# Autodesk Inventor assembly: Ball Intake
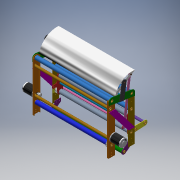
[picture p0: Inventor's stored thumbnail of the model, 180x180]
Saved by Autodesk Inventor 2017 (Build 210142000, 142)
## iProperties
Created: 2017-01-13
Part Number: Ball Intake
Document SubType Name: Assembly
Designer: Ben
Author: Ben
## Documents named in this file (27)
- C:\Users\Ben\Desktop\Projects\2017 Robot\Ball Intake\Ball Intake.iam
- C:\Users\Ben\Desktop\Projects\2017 Robot\Ball Intake\Front Plate.ipt
- C:\Users\Ben\Desktop\Projects\2017 Robot\Ball Intake\Churro Cross Brace.ipt
- C:\Users\Ben\Desktop\Projects\2017 Robot\Ball Intake\Back Plate.ipt
- C:\Users\Ben\Desktop\Projects\2017 Robot\Ball Intake\Cross Plate.ipt
- C:\Users\Ben\Desktop\Projects\2017 Robot\Ball Intake\Roller Assembly.iam
- C:\Users\Ben\Desktop\Projects\2017 Robot\Ball Intake\Swing Arm.ipt
- C:\Users\Ben\Desktop\Projects\2017 Robot\Ball Intake\Rear roller plate.ipt
- C:\Users\Ben\Desktop\Projects\2017 Robot\Ball Intake\Hopper pully plate.ipt
- C:\Users\Ben\Desktop\Projects\2017 Robot\Ball Intake\Flipper Plate.ipt
- C:\Users\Ben\Desktop\Projects\2017 Robot\Ball Intake\Kick Plate.ipt
- C:\Users\Ben\Desktop\Projects\2017 Robot\Ball Intake\Shorter Churro Cross Brace.ipt
- C:\Users\Ben\Desktop\Projects\2017 Robot\Ball Intake\Hopper roller assembly.iam
- C:\Users\Ben\Desktop\Projects\2017 Robot\Ball Intake\Hopper roller rear assembly.iam
- C:\Users\Ben\Desktop\Projects\2017 Robot\Ball Intake\Front Idler roller assembly.iam
- C:\Users\Ben\Desktop\Projects\2017 Robot\Ball Intake\Mini CIM.ipt
- C:\Users\Ben\Desktop\Projects\2017 Robot\Ball Intake\.375 bearing.ipt
- C:\Users\Ben\Desktop\Projects\2017 Robot\Ball Intake\Front C Left.ipt
- C:\Users\Ben\Desktop\Projects\2017 Robot\Ball Intake\.25 bushing.ipt
- C:\Users\Ben\Desktop\Projects\2017 Robot\Ball Intake\XL 24T Pulley.ipt
- C:\Users\Ben\Desktop\Projects\2017 Robot\Ball Intake\XL 12T Timing Pulley.ipt
- C:\Users\Ben\Desktop\Projects\2017 Robot\Ball Intake\1in Short PVC Roller.ipt
- C:\Users\Ben\Desktop\Projects\2017 Robot\Ball Intake\Bottom Roller.ipt
- C:\Users\Ben\Desktop\Projects\2017 Robot\Ball Intake\Roller End Plug.ipt
- C:\Users\Ben\Desktop\Projects\2017 Robot\Ball Intake\Intake Roller.ipt
- C:\Users\Ben\Desktop\Projects\2017 Robot\Ball Intake\Tie Rod 2.ipt
- C:\Users\Ben\Desktop\Projects\2017 Robot\Ball Intake\Cross Brace.ipt
## Components (73 placed, 26 different names)
1. Front Plate:2 — Flush:2, Insert:10, Flush:6, Flush:17, Flush:18, Mate:10, Insert:46, Insert:55, Insert:56, Insert:82, Mate:14, Flush:22, Flush:23, Insert:113, Mate:17, Angle:1
2. Back Plate:1 — Insert:5, Insert:13, Mate:3, Flush:8, Mate:6, Insert:28, Flush:9, Flush:19, Insert:130, Insert:131, Insert:142, Insert:143
3. Back Plate:2 — Flush:2, Insert:7, Flush:6, Insert:25, Mate:4, Flush:7, Mate:5, Insert:27, Flush:10, Flush:17, Flush:19, Insert:115, Insert:117, Insert:140, Insert:141
4. Churro Cross Brace:3 — Insert:5, Insert:7
5. Cross Plate:1 — Insert:10, Insert:25, Mate:7, Mate:12, Flush:20
6. Cross Plate:2 — Insert:13, Mate:8, Flush:21
7. Roller Assembly:4 [sub-assembly] — Insert:118
8. Swing Arm:1 — Insert:39, Insert:60, Insert:66, Insert:135, Insert:137, Angle:1, Insert:139
9. Swing Arm:2 — Insert:71, Insert:75
10. Rear roller plate:3 — Mate:3, Flush:8, Mate:6, Insert:67
11. Rear roller plate:4 — Mate:4, Flush:7, Mate:5, Insert:63
12. Hopper pully plate:1 — Insert:27, Flush:10, Insert:61, Insert:62, Insert:64
13. Hopper pully plate:2 — Insert:28, Flush:9, Insert:74, Insert:76, Insert:77
14. Flipper Plate:1 — Mate:7, Flush:14, Insert:31, Mate:12, Flush:20, Insert:89
15. Flipper Plate:2 — Mate:8, Flush:14, Flush:21, Insert:90
16. Kick Plate:1 — Insert:31, Mate:21, Insert:138
17. Shorter Churro Cross Brace:1 — Insert:39
18. Hopper roller assembly:1 [sub-assembly] — Insert:124
19. Hopper roller rear assembly:1 [sub-assembly] — Insert:123
20. Front Idler roller assembly:1 [sub-assembly] — Insert:133
21. Front Idler roller assembly:2 [sub-assembly] — Insert:122
22. Mini CIM:1 — Insert:46, Insert:94, Mate:17
23. Mini CIM:2 — Insert:87, Mate:15, Insert:95
24. Roller Assembly:5 [sub-assembly] — Insert:114
25. Roller Assembly:6 [sub-assembly] — Insert:116
26. .375 bearing:1 — Insert:63, Insert:128
27. .375 bearing:2 — Insert:55, Insert:93, Insert:121
28. .375 bearing:3 — Insert:56, Insert:122
29. .375 bearing:7 — Insert:64, Insert:123
30. .375 bearing:8 — Insert:60, Insert:132
31. .375 bearing:9 — Insert:61, Insert:135
32. .375 bearing:10 — Insert:62, Insert:124
33. .375 bearing:11 — Insert:66, Insert:127
34. .375 bearing:12 — Insert:67
35. .375 bearing:13 — Insert:84
36. .375 bearing:14 — Insert:83
37. .375 bearing:18 — Insert:77
38. .375 bearing:19 — Insert:76
39. .375 bearing:20 — Insert:74, Insert:109
40. .375 bearing:21 — Insert:75, Mate:20
41. .375 bearing:22 — Insert:71, Mate:18, Insert:136
42. .375 bearing:23 — Insert:85
43. .375 bearing:24 — Insert:82, Insert:133
44. Front C Left:1 — Mate:14, Flush:22, Flush:23, Insert:83, Insert:84, Insert:85, Insert:87, Mate:15, Insert:129
45. .25 bushing:1 — Insert:89
46. .25 bushing:2 — Insert:90
47. XL 24T Pulley:1 — Insert:93
48. XL 12T Timing Pulley:1 — Insert:94
49. XL 12T Timing Pulley:2 — Insert:95
50. 1in Short PVC Roller:1 — Insert:125, Insert:126
51. Bottom Roller:1 — Insert:99, Insert:100
52. Roller End Plug:1 — Insert:99
53. Roller End Plug:2 — Insert:100, Insert:128
54. 1in Short PVC Roller:2 — Insert:102, Insert:103
55. Roller End Plug:3 — Insert:102, Insert:132
56. Roller End Plug:4 — Insert:103, Mate:18, Insert:136
57. XL 24T Pulley:2 — Insert:109
58. .375 bearing:25 — Insert:113, Insert:114
59. .375 bearing:26 — Insert:115, Insert:116
60. .375 bearing:27 — Insert:117, Insert:118
61. Intake Roller:1 — Insert:119, Insert:120
62. Roller End Plug:5 — Insert:119, Insert:121
63. Roller End Plug:6 — Insert:120
64. Roller End Plug:7 — Insert:125, Mate:20
65. Roller End Plug:8 — Insert:126, Insert:127
66. .375 bearing:28 — Insert:129
67. .375 bearing:29 — Insert:130
68. .375 bearing:30 — Insert:131
69. Tie Rod 2:1 — Insert:137, Mate:21
70. .25 bushing:3 — Insert:138
71. .25 bushing:4 — Insert:139
72. Cross Brace:1 — Insert:140, Insert:141
73. Cross Brace:2 — Insert:142, Insert:143
## Relationships (98: Insert 69, Flush 14, Mate 14, Angle 1)
- Flush:2: Front Plate:2 ↔ Back Plate:2
- Insert:5: Back Plate:1 ↔ Churro Cross Brace:3
- Insert:7: Back Plate:2 ↔ Churro Cross Brace:3
- Insert:10: Front Plate:2 ↔ Cross Plate:1
- Insert:13: Back Plate:1 ↔ Cross Plate:2
- Flush:6: Front Plate:2 ↔ Back Plate:2
- Insert:25: Back Plate:2 ↔ Cross Plate:1
- Mate:3 (12.7 mm): Back Plate:1 ↔ Rear roller plate:3
- Mate:4 (12.7 mm): Back Plate:2 ↔ Rear roller plate:4
- Flush:7: Back Plate:2 ↔ Rear roller plate:4
- Mate:5: Back Plate:2 ↔ Rear roller plate:4
- Flush:8: Back Plate:1 ↔ Rear roller plate:3
- Mate:6: Back Plate:1 ↔ Rear roller plate:3
- Insert:27: Back Plate:2 ↔ Hopper pully plate:1
- Insert:28: Back Plate:1 ↔ Hopper pully plate:2
- Flush:9: Back Plate:1 ↔ Hopper pully plate:2
- Flush:10: Back Plate:2 ↔ Hopper pully plate:1
- Mate:7: Cross Plate:1 ↔ Flipper Plate:1
- Mate:8: Cross Plate:2 ↔ Flipper Plate:2
- Flush:14: Flipper Plate:1 ↔ Flipper Plate:2
- Insert:31 (3.175 mm): Flipper Plate:1 ↔ Kick Plate:1
- Flush:17: Front Plate:2 ↔ Back Plate:2
- Flush:18 (53.975 mm): Front Plate:2
- Mate:10 (57.658 mm): Front Plate:2
- Flush:19: Back Plate:1 ↔ Back Plate:2
- Insert:39: Swing Arm:1 ↔ Shorter Churro Cross Brace:1
- Mate:12 (61.9252 mm): Cross Plate:1 ↔ Flipper Plate:1
- Insert:46 (2.3622 mm): Front Plate:2 ↔ Mini CIM:1
- Insert:55: Front Plate:2 ↔ .375 bearing:2
- Insert:56: Front Plate:2 ↔ .375 bearing:3
- Insert:60: Swing Arm:1 ↔ .375 bearing:8
- Insert:61: Hopper pully plate:1 ↔ .375 bearing:9
- Insert:62: Hopper pully plate:1 ↔ .375 bearing:10
- Insert:63: Rear roller plate:4 ↔ .375 bearing:1
- Insert:64: Hopper pully plate:1 ↔ .375 bearing:7
- Insert:66: Swing Arm:1 ↔ .375 bearing:11
- Insert:67: Rear roller plate:3 ↔ .375 bearing:12
- Insert:71: Swing Arm:2 ↔ .375 bearing:22
- Insert:74: Hopper pully plate:2 ↔ .375 bearing:20
- Insert:75: Swing Arm:2 ↔ .375 bearing:21
- Insert:76: Hopper pully plate:2 ↔ .375 bearing:19
- Insert:77: Hopper pully plate:2 ↔ .375 bearing:18
- Insert:82: Front Plate:2 ↔ .375 bearing:24
- Flush:20: Cross Plate:1 ↔ Flipper Plate:1
- Flush:21: Cross Plate:2 ↔ Flipper Plate:2
- Mate:14 (-615.95 mm): Front Plate:2 ↔ Front C Left:1
- Flush:22: Front Plate:2 ↔ Front C Left:1
- Flush:23: Front Plate:2 ↔ Front C Left:1
- Insert:83: .375 bearing:14 ↔ Front C Left:1
- Insert:84: .375 bearing:13 ↔ Front C Left:1
- Insert:85: .375 bearing:23 ↔ Front C Left:1
- Insert:87 (2.3622 mm): Mini CIM:2 ↔ Front C Left:1
- Mate:15: Mini CIM:2 ↔ Front C Left:1
- Insert:89: Flipper Plate:1 ↔ .25 bushing:1
- Insert:90: Flipper Plate:2 ↔ .25 bushing:2
- Insert:93 (1.5875 mm): .375 bearing:2 ↔ XL 24T Pulley:1
- Insert:94 (1.5875 mm): Mini CIM:1 ↔ XL 12T Timing Pulley:1
- Insert:95 (6.35 mm): Mini CIM:2 ↔ XL 12T Timing Pulley:2
- Insert:99: Bottom Roller:1 ↔ Roller End Plug:1
- Insert:100: Bottom Roller:1 ↔ Roller End Plug:2
- Insert:102: 1in Short PVC Roller:2 ↔ Roller End Plug:3
- Insert:103: 1in Short PVC Roller:2 ↔ Roller End Plug:4
- Insert:109 (1.5875 mm): .375 bearing:20 ↔ XL 24T Pulley:2
- Insert:113: Front Plate:2 ↔ .375 bearing:25
- Insert:114 (1.5875 mm): Roller Assembly:5 ↔ .375 bearing:25
- Insert:115: Back Plate:2 ↔ .375 bearing:26
- Insert:116 (1.5875 mm): Roller Assembly:6 ↔ .375 bearing:26
- Insert:117: Back Plate:2 ↔ .375 bearing:27
- Insert:118 (1.5875 mm): Roller Assembly:4 ↔ .375 bearing:27
- Insert:119: Intake Roller:1 ↔ Roller End Plug:5
- Insert:120: Intake Roller:1 ↔ Roller End Plug:6
- Insert:121 (22.225 mm): .375 bearing:2 ↔ Roller End Plug:5
- Insert:122 (1.5875 mm): Front Idler roller assembly:2 ↔ .375 bearing:3
- Insert:123 (1.5875 mm): Hopper roller rear assembly:1 ↔ .375 bearing:7
- Mate:17: Front Plate:2 ↔ Mini CIM:1
- Insert:124 (1.5875 mm): Hopper roller assembly:1 ↔ .375 bearing:10
- Insert:125: 1in Short PVC Roller:1 ↔ Roller End Plug:7
- Insert:126: 1in Short PVC Roller:1 ↔ Roller End Plug:8
- Insert:127 (1.5875 mm): .375 bearing:11 ↔ Roller End Plug:8
- Insert:128 (1.5875 mm): .375 bearing:1 ↔ Roller End Plug:2
- Insert:129: Front C Left:1 ↔ .375 bearing:28
- Insert:130: Back Plate:1 ↔ .375 bearing:29
- Insert:131: Back Plate:1 ↔ .375 bearing:30
- Mate:18: .375 bearing:22 ↔ Roller End Plug:4
- Insert:132 (1.5875 mm): .375 bearing:8 ↔ Roller End Plug:3
- Insert:133 (1.5875 mm): Front Idler roller assembly:1 ↔ .375 bearing:24
- Insert:135 (3.175 mm): Swing Arm:1 ↔ .375 bearing:9
- Insert:136 (1.5875 mm): .375 bearing:22 ↔ Roller End Plug:4
- Mate:20: .375 bearing:21 ↔ Roller End Plug:7
- Insert:137 (1.5875 mm): Swing Arm:1 ↔ Tie Rod 2:1
- Mate:21: Kick Plate:1 ↔ Tie Rod 2:1
- Angle:1 (-70 deg): Front Plate:2 ↔ Swing Arm:1
- Insert:138: Kick Plate:1 ↔ .25 bushing:3
- Insert:139: Swing Arm:1 ↔ .25 bushing:4
- Insert:140: Back Plate:2 ↔ Cross Brace:1
- Insert:141: Back Plate:2 ↔ Cross Brace:1
- Insert:142: Back Plate:1 ↔ Cross Brace:2
- Insert:143: Back Plate:1 ↔ Cross Brace:2
